# Autodesk Inventor assembly: Assembly1
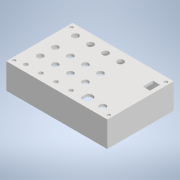
[picture p0: Inventor's stored thumbnail of the model, 180x180]
Saved by Autodesk Inventor 2022 (Build 260153000, 153)
## iProperties
Created: 2021-07-28
Part Number: Assembly1
Document SubType Name: Assembly
Designer: Matthijs
Author: Matthijs
## Documents named in this file (3)
- C:\Users\Matthijs\Documents\Main_Files\DIY\ButtonBox 3D Parts\Assembly1.iam
- C:\Users\Matthijs\Documents\Main_Files\DIY\ButtonBox 3D Parts\Box Top.ipt
- C:\Users\Matthijs\Documents\Main_Files\DIY\ButtonBox 3D Parts\Box2.ipt
## Components (2 placed, 2 different names)
1. Box Top:1 — Mate:1, Flush:1, Mate:2, Flush:2
2. Box2:1 — Mate:1, Flush:1, Mate:2, Flush:2
## Relationships (4: Mate 2, Flush 2)
- Mate:1: Box Top:1 ↔ Box2:1
- Flush:1: Box Top:1 ↔ Box2:1
- Mate:2: Box Top:1 ↔ Box2:1
- Flush:2: Box Top:1 ↔ Box2:1
